# Autodesk Inventor assembly: Full_Assembly
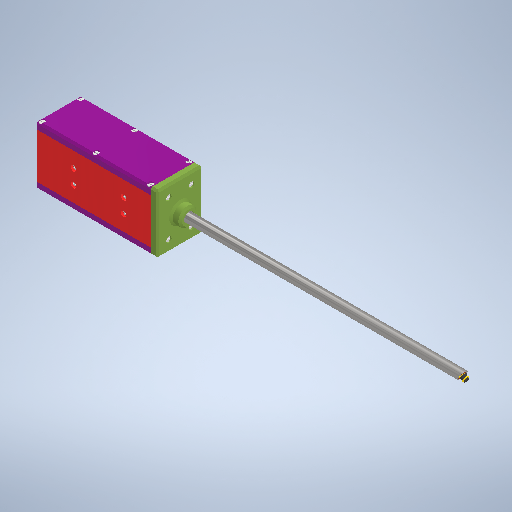
[picture p0: Inventor's stored thumbnail of the model, 512x512]
Saved by Autodesk Inventor 2026.2 (Build 302298010, 298A)
## iProperties
Created: 2026-05-14
Part Number: Full_Assembly
Document SubType Name: Assembly
Designer: piete
Author: piete
## Documents named in this file (5)
- C:\Users\piete\Desktop\Skripsie\Documents\Detail Design\Full_Assembly.iam
- C:\Users\piete\Desktop\Skripsie\Documents\Detail Design\Main Body Design\Main_Body_Assembly.iam
- C:\Users\piete\Desktop\Skripsie\Documents\Detail Design\Handle Design\Handle_Assembly.iam
- C:\Users\piete\OneDrive\Documents\Inventor\Content Center Files\R2026\en-US\ISO 2009(2)\ISO 2009 - M2 x 16 - 14 - ISO.ipt
- C:\Users\piete\OneDrive\Documents\Inventor\Content Center Files\R2026\en-US\ISO 4036(2)\ISO 4036 - M2(2).ipt
## Components (26 placed, 4 different names)
1. Main_Body_Assembly:1 [sub-assembly] — Mate:1, Mate:2, Mate:3, Mate:13, Mate:15, Mate:17, Mate:19, Mate:21, Mate:23, Mate:25, Mate:27, Flush:13, Flush:14, Flush:15, Flush:16, Flush:17, Flush:18, Flush:19, Angle:5, Angle:6, Angle:7, Angle:8
2. Handle_Assembly:1 [sub-assembly] — Mate:1, Mate:2, Mate:3, Mate:4, Flush:1, Mate:5, Mate:6, Mate:7, Flush:4, Angle:1, Angle:2, Mate:8, Mate:9, Mate:10, Mate:11, Flush:10, Angle:3, Angle:4
3. ISO 2009 M2 x 16 x 14:1 — Mate:4, Flush:1, Flush:5, Mate:14, Mate:33
4. ISO 2009 M2 x 16 x 14:2 — Flush:2, Flush:3, Mate:7, Flush:6, Angle:1, Mate:26, Mate:28
5. ISO 2009 M2 x 16 x 14:3 — Flush:3, Mate:5, Flush:4, Flush:5, Angle:2, Mate:12, Mate:34
6. ISO 2009 M2 x 16 x 14:4 — Flush:2, Mate:6, Flush:6, Mate:24, Mate:31, Mate:32
7. ISO 2009 M2 x 16 x 14:5 — Flush:8, Flush:9, Mate:10, Flush:11, Mate:16, Mate:36
8. ISO 2009 M2 x 16 x 14:6 — Flush:7, Flush:9, Mate:11, Flush:10, Flush:11, Angle:4, Mate:18, Mate:35
9. ISO 2009 M2 x 16 x 14:7 — Flush:8, Mate:9, Flush:12, Mate:22, Mate:30
10. ISO 2009 M2 x 16 x 14:8 — Flush:7, Mate:8, Flush:12, Angle:3, Mate:20, Mate:29
11. ISO 4036 M2:1 — Mate:12, Mate:13, Flush:20, Flush:25, Angle:6
12. ISO 4036 M2:2 — Mate:14, Mate:15, Flush:21, Flush:23, Angle:5
13. ISO 4036 M2:3 — Mate:16, Mate:17, Flush:29, Flush:31
14. ISO 4036 M2:4 — Mate:18, Mate:19, Flush:26, Flush:28, Angle:7
15. ISO 4036 M2:5 — Mate:20, Mate:21, Flush:27, Flush:28
16. ISO 4036 M2:6 — Mate:22, Mate:23, Flush:30, Flush:31, Angle:8
17. ISO 4036 M2:7 — Mate:24, Mate:25, Flush:21, Flush:22
18. ISO 4036 M2:8 — Mate:26, Mate:27, Flush:20, Flush:24
19. ISO 4036 M2:9 — Mate:28, Flush:19, Flush:24
20. ISO 4036 M2:10 — Mate:29, Flush:18, Flush:27
21. ISO 4036 M2:11 — Mate:30, Flush:17, Flush:30
22. ISO 4036 M2:12 — Mate:31, Mate:32, Flush:22
23. ISO 4036 M2:13 — Mate:33, Flush:13, Flush:23
24. ISO 4036 M2:14 — Mate:34, Flush:14, Flush:25
25. ISO 4036 M2:15 — Mate:35, Flush:15, Flush:26
26. ISO 4036 M2:16 — Mate:36, Flush:16, Flush:29
## Relationships (75: Mate 36, Flush 31, Angle 8)
- Mate:1: Main_Body_Assembly:1 ↔ Handle_Assembly:1
- Mate:2: Main_Body_Assembly:1 ↔ Handle_Assembly:1
- Mate:3: Main_Body_Assembly:1 ↔ Handle_Assembly:1
- Mate:4: Handle_Assembly:1 ↔ ISO 2009 M2 x 16 x 14:1
- Flush:1 (1.5 mm): Handle_Assembly:1 ↔ ISO 2009 M2 x 16 x 14:1
- Flush:2: ISO 2009 M2 x 16 x 14:2 ↔ ISO 2009 M2 x 16 x 14:4
- Flush:3: ISO 2009 M2 x 16 x 14:2 ↔ ISO 2009 M2 x 16 x 14:3
- Mate:5: Handle_Assembly:1 ↔ ISO 2009 M2 x 16 x 14:3
- Mate:6: Handle_Assembly:1 ↔ ISO 2009 M2 x 16 x 14:4
- Mate:7: Handle_Assembly:1 ↔ ISO 2009 M2 x 16 x 14:2
- Flush:4 (1.5 mm): Handle_Assembly:1 ↔ ISO 2009 M2 x 16 x 14:3
- Flush:5: ISO 2009 M2 x 16 x 14:1 ↔ ISO 2009 M2 x 16 x 14:3
- Flush:6: ISO 2009 M2 x 16 x 14:2 ↔ ISO 2009 M2 x 16 x 14:4
- Angle:1 (90 deg): Handle_Assembly:1 ↔ ISO 2009 M2 x 16 x 14:2
- Angle:2 (90 deg): Handle_Assembly:1 ↔ ISO 2009 M2 x 16 x 14:3
- Flush:7: ISO 2009 M2 x 16 x 14:6 ↔ ISO 2009 M2 x 16 x 14:8
- Flush:8: ISO 2009 M2 x 16 x 14:5 ↔ ISO 2009 M2 x 16 x 14:7
- Flush:9: ISO 2009 M2 x 16 x 14:5 ↔ ISO 2009 M2 x 16 x 14:6
- Mate:8: Handle_Assembly:1 ↔ ISO 2009 M2 x 16 x 14:8
- Mate:9: Handle_Assembly:1 ↔ ISO 2009 M2 x 16 x 14:7
- Mate:10: Handle_Assembly:1 ↔ ISO 2009 M2 x 16 x 14:5
- Mate:11: Handle_Assembly:1 ↔ ISO 2009 M2 x 16 x 14:6
- Flush:10 (1.5 mm): Handle_Assembly:1 ↔ ISO 2009 M2 x 16 x 14:6
- Flush:11: ISO 2009 M2 x 16 x 14:5 ↔ ISO 2009 M2 x 16 x 14:6
- Flush:12: ISO 2009 M2 x 16 x 14:7 ↔ ISO 2009 M2 x 16 x 14:8
- Angle:3 (90 deg): Handle_Assembly:1 ↔ ISO 2009 M2 x 16 x 14:8
- Angle:4 (90 deg): Handle_Assembly:1 ↔ ISO 2009 M2 x 16 x 14:6
- Mate:12: ISO 2009 M2 x 16 x 14:3 ↔ ISO 4036 M2:1
- Mate:13: Main_Body_Assembly:1 ↔ ISO 4036 M2:1
- Mate:14: ISO 2009 M2 x 16 x 14:1 ↔ ISO 4036 M2:2
- Mate:15: Main_Body_Assembly:1 ↔ ISO 4036 M2:2
- Mate:16: ISO 2009 M2 x 16 x 14:5 ↔ ISO 4036 M2:3
- Mate:17: Main_Body_Assembly:1 ↔ ISO 4036 M2:3
- Mate:18: ISO 2009 M2 x 16 x 14:6 ↔ ISO 4036 M2:4
- Mate:19: Main_Body_Assembly:1 ↔ ISO 4036 M2:4
- Mate:20: ISO 2009 M2 x 16 x 14:8 ↔ ISO 4036 M2:5
- Mate:21: Main_Body_Assembly:1 ↔ ISO 4036 M2:5
- Mate:22: ISO 2009 M2 x 16 x 14:7 ↔ ISO 4036 M2:6
- Mate:23: Main_Body_Assembly:1 ↔ ISO 4036 M2:6
- Mate:24: ISO 2009 M2 x 16 x 14:4 ↔ ISO 4036 M2:7
- Mate:25: Main_Body_Assembly:1 ↔ ISO 4036 M2:7
- Mate:26: ISO 2009 M2 x 16 x 14:2 ↔ ISO 4036 M2:8
- Mate:27: Main_Body_Assembly:1 ↔ ISO 4036 M2:8
- Mate:28: ISO 2009 M2 x 16 x 14:2 ↔ ISO 4036 M2:9
- Mate:29: ISO 2009 M2 x 16 x 14:8 ↔ ISO 4036 M2:10
- Mate:30: ISO 2009 M2 x 16 x 14:7 ↔ ISO 4036 M2:11
- Mate:31: ISO 2009 M2 x 16 x 14:4 ↔ ISO 4036 M2:12
- Mate:32: ISO 2009 M2 x 16 x 14:4 ↔ ISO 4036 M2:12
- Mate:33: ISO 2009 M2 x 16 x 14:1 ↔ ISO 4036 M2:13
- Mate:34: ISO 2009 M2 x 16 x 14:3 ↔ ISO 4036 M2:14
- Mate:35: ISO 2009 M2 x 16 x 14:6 ↔ ISO 4036 M2:15
- Mate:36: ISO 2009 M2 x 16 x 14:5 ↔ ISO 4036 M2:16
- Flush:13 (1.4 mm): Main_Body_Assembly:1 ↔ ISO 4036 M2:13
- Flush:14 (1.4 mm): Main_Body_Assembly:1 ↔ ISO 4036 M2:14
- Flush:15 (-1.4 mm): Main_Body_Assembly:1 ↔ ISO 4036 M2:15
- Flush:16 (1.4 mm): Main_Body_Assembly:1 ↔ ISO 4036 M2:16
- Flush:17 (1.4 mm): Main_Body_Assembly:1 ↔ ISO 4036 M2:11
- Flush:18 (1.4 mm): Main_Body_Assembly:1 ↔ ISO 4036 M2:10
- Flush:19 (-1.4 mm): Main_Body_Assembly:1 ↔ ISO 4036 M2:9
- Flush:20: ISO 4036 M2:1 ↔ ISO 4036 M2:8
- Flush:21: ISO 4036 M2:2 ↔ ISO 4036 M2:7
- Flush:22: ISO 4036 M2:7 ↔ ISO 4036 M2:12
- Flush:23: ISO 4036 M2:2 ↔ ISO 4036 M2:13
- Angle:5 (0 deg): Main_Body_Assembly:1 ↔ ISO 4036 M2:2
- Flush:24: ISO 4036 M2:8 ↔ ISO 4036 M2:9
- Flush:25: ISO 4036 M2:1 ↔ ISO 4036 M2:14
- Angle:6 (0 deg): Main_Body_Assembly:1 ↔ ISO 4036 M2:1
- Flush:26: ISO 4036 M2:4 ↔ ISO 4036 M2:15
- Flush:27: ISO 4036 M2:5 ↔ ISO 4036 M2:10
- Flush:28: ISO 4036 M2:4 ↔ ISO 4036 M2:5
- Angle:7 (0 deg): Main_Body_Assembly:1 ↔ ISO 4036 M2:4
- Flush:29: ISO 4036 M2:3 ↔ ISO 4036 M2:16
- Flush:30: ISO 4036 M2:6 ↔ ISO 4036 M2:11
- Flush:31: ISO 4036 M2:3 ↔ ISO 4036 M2:6
- Angle:8 (0 deg): Main_Body_Assembly:1 ↔ ISO 4036 M2:6
